# Autodesk Inventor assembly: Storage System Assembly
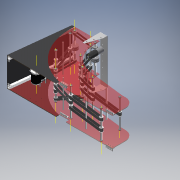
[picture p0: Inventor's stored thumbnail of the model, 180x180]
Saved by Autodesk Inventor 2019.4 (Build 234330000, 330)
## iProperties
Created: 2020-01-11
Part Number: Storage System Assembly
Document SubType Name: Assembly
Designer: admin
Mass: 8566.96 g
Surface Area: 28406.6 cm^2
Volume: 5013.1 cm^3
Density: 1.70891 g/cm^3
Author: admin
## Documents named in this file (37)
- C:\Users\admin\Desktop\FRC 2020 Engineering\GitHub\7738-2020\Storage system\Storage System Assembly.iam
- C:\Users\admin\Desktop\FRC 2020 Engineering\GitHub\7738-2020\Storage system\Turret Base Plate.ipt
- C:\Users\admin\Desktop\FRC 2020 Engineering\GitHub\7738-2020\Storage system\Storage Side Plate.ipt
- C:\Users\admin\Desktop\FRC 2020 Engineering\GitHub\7738-2020\CAD\Gearbox\F6800.ipt
- C:\Users\admin\Desktop\FRC 2020 Engineering\GitHub\7738-2020\Storage system\Storage System Assembly\Design Accelerator\Synchronous Belts Transmission1.iam
- C:\Users\admin\Desktop\FRC 2020 Engineering\GitHub\7738-2020\Storage system\Storage System Assembly\Design Accelerator\Synchronous Belts Transmission2.iam
- C:\Users\admin\Desktop\FRC 2020 Engineering\GitHub\7738-2020\Storage system\Storage System Assembly\Design Accelerator\Synchronous Belts Transmission3.iam
- C:\Users\admin\Desktop\FRC 2020 Engineering\GitHub\7738-2020\Storage system\Storage System Assembly\Design Accelerator\Synchronous Belts Transmission5.iam
- C:\Users\admin\Desktop\FRC 2020 Engineering\GitHub\7738-2020\Storage system\Storage System Assembly\Design Accelerator\Synchronous Belts Transmission6.iam
- C:\Users\admin\Desktop\FRC 2020 Engineering\GitHub\7738-2020\Storage system\Storage System Assembly\Design Accelerator\Synchronous Belts Transmission7.iam
- C:\Users\admin\Desktop\FRC 2020 Engineering\GitHub\7738-2020\Storage system\Storage System Assembly\Design Accelerator\Synchronous Belts Transmission8.iam
- C:\Users\admin\Desktop\FRC 2020 Engineering\GitHub\7738-2020\Storage system\Storage System Assembly\Design Accelerator\Synchronous Belts Transmission9.iam
- C:\Users\admin\Desktop\FRC 2020 Engineering\GitHub\7738-2020\Storage system\Complaint Wheel.ipt
- C:\Users\admin\Desktop\FRC 2020 Engineering\GitHub\7738-2020\Storage system\Belt Axle.ipt
- C:\Users\admin\Desktop\FRC 2020 Engineering\GitHub\7738-2020\Storage system\Storage System Assembly\Design Accelerator\Synchronous Belts Transmission4.iam
- C:\Users\admin\Desktop\FRC 2020 Engineering\GitHub\7738-2020\Storage system\Storage System Assembly\Design Accelerator\Synchronous Belts Transmission10.iam
- C:\Users\admin\Desktop\FRC 2020 Engineering\GitHub\7738-2020\Storage system\Storage System Assembly\Design Accelerator\Synchronous Belts Transmission11.iam
- C:\Users\admin\Desktop\FRC 2020 Engineering\GitHub\7738-2020\Storage system\Storage System Assembly\Design Accelerator\Synchronous Belts Transmission12.iam
- C:\Users\admin\Desktop\FRC 2020 Engineering\GitHub\7738-2020\Storage system\Storage Plate Spacer.ipt
- C:\Users\admin\Desktop\FRC 2020 Engineering\GitHub\7738-2020\Storage system\PC Plate Bracket.ipt
- C:\Users\admin\Desktop\FRC 2020 Engineering\GitHub\7738-2020\Storage system\Turret Support Extrusion.ipt
- C:\Users\admin\Desktop\FRC 2020 Engineering\GitHub\7738-2020\Storage system\Back PC Cover.ipt
- C:\Users\admin\Desktop\FRC 2020 Engineering\GitHub\7738-2020\Storage system\Side CFRP Cover.ipt
- C:\Users\admin\Desktop\FRC 2020 Engineering\GitHub\7738-2020\Storage system\Turret Drive Gear.ipt
- C:\Users\admin\Desktop\FRC 2020 Engineering\GitHub\7738-2020\Storage system\Sport Gearbox\775pro_217-4347.ipt
- C:\Users\admin\Desktop\FRC 2020 Engineering\GitHub\7738-2020\Storage system\775 16 reduction Gearbox.ipt
- C:\Users\admin\Desktop\FRC 2020 Engineering\GitHub\7738-2020\Turret\Turret Support Brace.ipt
- C:\Users\admin\Desktop\FRC 2020 Engineering\GitHub\7738-2020\Storage system\Brace.ipt
- C:\Users\admin\Desktop\FRC 2020 Engineering\GitHub\7738-2020\Storage system\Intake Motor Mount.ipt
- C:\Users\admin\Desktop\FRC 2020 Engineering\GitHub\7738-2020\Turret\Mini CIM\Mini_CIM_Motor_217-3371.ipt
- C:\Users\admin\Desktop\FRC 2020 Engineering\GitHub\7738-2020\Storage system\Storage System Assembly\Design Accelerator\Synchronous Belts Transmission13.iam
- C:\Users\admin\Desktop\FRC 2020 Engineering\GitHub\7738-2020\Storage system\Spacer.ipt
- C:\Users\admin\Desktop\FRC 2020 Engineering\GitHub\7738-2020\Storage system\Storage System Assembly\Design Accelerator\Synchronous Belts Transmission14.iam
- C:\Users\admin\Desktop\FRC 2020 Engineering\GitHub\7738-2020\Storage system\Storage System Assembly\Design Accelerator\Synchronous Belts Transmission15.iam
- C:\Users\admin\Desktop\FRC 2020 Engineering\GitHub\7738-2020\Storage system\Storage Shooter Axle.ipt
- C:\Users\admin\Desktop\FRC 2020 Engineering\GitHub\7738-2020\Storage system\Storage System Assembly\Design Accelerator\Spur Gears1.iam
- C:\Users\admin\Desktop\FRC 2020 Engineering\GitHub\7738-2020\Storage system\Storage System Assembly\Design Accelerator\Synchronous Belts Transmission16.iam
## Components (98 placed, 21 different names)
1. Turret Base Plate:1 — Mate:1, Mate:3, Mate:4, Flush:1, Mate:5, Mate:8, Mate:9, Angle:1, Mate:107, Mate:108, Mate:110, Mate:119, Mate:120, Mate:121, Mate:122, Mate:125, Mate:126, Flush:16, Mate:132, Mate:135
2. Storage Side Plate:1 — Mate:1, Mate:7, Mate:8, Mate:10, Mate:11, Mate:12, Mate:13, Mate:14, Mate:15, Mate:16, Mate:17, Mate:18, Mate:19, Mate:20, Mate:21, Mate:22, Mate:23, Mate:24, Mate:25, Mate:26, Mate:27, Mate:28, Mate:29, Mate:30, Mate:31, Mate:32, Mate:33, Symmetry:1, Mate:75, Mate:93, Mate:94, Mate:95, Mate:96, Mate:97, Mate:98, Mate:99, Mate:100, Mate:101, Flush:4, Mate:102, Mate:105, Flush:6, Flush:7, Mate:107, Mate:111, Flush:11, Mate:114, Mate:115, Flush:12, Flush:13, Mate:137, Mate:138, Mate:139, Mate:147, Mate:148, Mate:149, Mate:150, Mate:169, Mate:170, Mate:171
3. Storage Side Plate:2 — Mate:5, Mate:7, Mate:9, Symmetry:1, Mate:41, Mate:42, Mate:43, Mate:44, Mate:45, Mate:46, Mate:47, Mate:48, Mate:49, Mate:50, Mate:51, Mate:52, Mate:53, Mate:54, Mate:55, Mate:56, Mate:57, Mate:58, Mate:59, Mate:60, Mate:61, Mate:62, Mate:63, Mate:64, Mate:85, Mate:86, Mate:87, Mate:88, Mate:89, Mate:90, Mate:91, Mate:92, Mate:103, Mate:104, Flush:5, Mate:106, Flush:8, Flush:9, Mate:109, Flush:10, Mate:113, Mate:116, Flush:14, Flush:15, Mate:157, Mate:162, Mate:163
4. Synchronous Belts Transmission:1 [sub-assembly] — Mate:66
5. Synchronous Belts Transmission:2 [sub-assembly]
6. Synchronous Belts Transmission:3 [sub-assembly]
7. Synchronous Belts Transmission:4 [sub-assembly]
8. Synchronous Belts Transmission:5 [sub-assembly]
9. Synchronous Belts Transmission:6 [sub-assembly]
10. Synchronous Belts Transmission:7 [sub-assembly]
11. Synchronous Belts Transmission:8 [sub-assembly]
12. F6800:11 — Mate:30, Mate:32, Mate:34
13. F6800:12 — Mate:31, Mate:33, Mate:39
14. Complaint Wheel:1 — Mate:34, Mate:35, Mate:36, Flush:3
15. Complaint Wheel:2 — Mate:35, Mate:36, Mate:40
16. Complaint Wheel:3 — Flush:3
17. Complaint Wheel:4 — Mate:39
18. Synchronous Belts Transmission:9 [sub-assembly]
19. Synchronous Belts Transmission:10 [sub-assembly]
20. Synchronous Belts Transmission:11 [sub-assembly]
21. Synchronous Belts Transmission:12 [sub-assembly]
22. Storage Plate Spacer:1 — Mate:85, Mate:93
23. Storage Plate Spacer:2 — Mate:89, Mate:100
24. Storage Plate Spacer:3 — Mate:90, Mate:99
25. Storage Plate Spacer:4 — Mate:91, Mate:98
26. Storage Plate Spacer:5 — Mate:92, Mate:97
27. Storage Plate Spacer:6 — Mate:88, Mate:96
28. Storage Plate Spacer:7 — Mate:87, Mate:95
29. Storage Plate Spacer:8 — Mate:86, Mate:94
30. PC Plate Bracket:1 — Mate:101, Flush:4, Mate:102
31. PC Plate Bracket:2 — Mate:103, Mate:104, Flush:5
32. PC Plate Bracket:3 — Mate:105, Flush:6, Flush:7
33. PC Plate Bracket:4 — Mate:106, Flush:8, Flush:9
34. Turret Support Extrusion:1 — Mate:108, Mate:109, Flush:10, Mate:112, Mate:127, Flush:17, Mate:128, Mate:131, Mate:133
35. Turret Support Extrusion:2 — Mate:110, Mate:111, Flush:11, Mate:129, Flush:18, Mate:130, Mate:134, Mate:136
36. Back PC Cover:1 — Mate:112, Mate:113, Mate:114
37. Side CFRP Cover:1 — Mate:115, Flush:12, Flush:13
38. Side CFRP Cover:2 — Mate:116, Flush:14, Flush:15
39. Turret Drive Gear:1 — Mate:119, Mate:120
40. 775pro_217-4347:1 — Mate:123, Mate:124
41. 775 16 reduction Gearbox:1 — Mate:121, Mate:122, Mate:123, Mate:124
42. Turret Support Brace:1 — Mate:125, Mate:126, Flush:16
43. Brace:1 — Mate:127, Flush:17, Mate:128
44. Brace:2 — Mate:129, Flush:18, Mate:130
45. Brace:3 — Mate:131, Mate:132, Mate:133
46. Brace:4 — Mate:134, Mate:135, Mate:136
47. Intake Motor Mount:1 — Mate:137, Mate:138, Mate:139, Mate:140, Mate:142, Mate:143, Mate:144, Mate:145, Mate:146
48. Mini_CIM_Motor_217-3371:1 — Mate:140, Mate:142
49. Synchronous Belts Transmission:13 [sub-assembly]
50. Spacer:1 — Mate:143, Mate:150
51. Spacer:2 — Mate:146, Mate:149
52. Spacer:3 — Mate:144, Mate:147
53. Spacer:4 — Mate:145, Mate:148
54. Synchronous Belts Transmission:14 [sub-assembly]
55. Intake Motor Mount:2 — Mate:157, Mate:158, Mate:159, Mate:160, Mate:161
56. Mini_CIM_Motor_217-3371:2
57. Spacer:5 — Mate:160
58. Spacer:6 — Mate:161
59. Spacer:7 — Mate:158, Mate:163
60. Spacer:8 — Mate:159, Mate:162
61. Synchronous Belts Transmission:15 [sub-assembly]
62. Storage Shooter Axle:1 — Mate:166, Mate:167, Mate:168
63. Storage Shooter Axle:2 — Mate:164, Mate:165
64. Spur Gears:1 [sub-assembly] — Mate:168, Mate:169
65. Synchronous Belts Transmission:16 [sub-assembly]
66. F6800:25 — Mate:170, Mate:171
67. Belt Axle:10 — Mate:74, Mate:84
68. Belt Axle:9 — Mate:73, Mate:83
69. Belt Axle:8 — Mate:72, Mate:82
70. Belt Axle:7 — Mate:71, Mate:81
71. Belt Axle:6 — Mate:70, Mate:80
72. Belt Axle:5 — Mate:69, Mate:75
73. Belt Axle:4 — Mate:68, Mate:76
74. Belt Axle:3 — Mate:67, Mate:77
75. Belt Axle:2 — Mate:66, Mate:78
76. Belt Axle:1 — Mate:65, Mate:79
77. F6800:10 — Mate:19, Mate:25, Mate:70, Mate:80
78. F6800:9 — Mate:18, Mate:26, Mate:71, Mate:81
79. F6800:7 — Mate:16, Mate:28, Mate:73, Mate:83
80. F6800:8 — Mate:17, Mate:27, Mate:72, Mate:82
81. F6800:6 — Mate:15, Mate:29, Mate:74, Mate:84
82. F6800:5 — Mate:14, Mate:24, Mate:69
83. F6800:4 — Mate:13, Mate:23, Mate:68, Mate:76
84. F6800:3 — Mate:12, Mate:22, Mate:67, Mate:77
85. F6800:2 — Mate:11, Mate:21, Mate:78
86. F6800:1 — Mate:10, Mate:20, Mate:65, Mate:79
87. F6800:24 — Mate:52, Mate:64
88. F6800:23 — Mate:51, Mate:63
89. F6800:22 — Mate:49, Mate:61
90. F6800:21 — Mate:50, Mate:62
91. F6800:20 — Mate:48, Mate:60
92. F6800:19 — Mate:47, Mate:59
93. F6800:18 — Mate:46, Mate:57
94. F6800:17 — Mate:45, Mate:58
95. F6800:16 — Mate:44, Mate:55
96. F6800:15 — Mate:42, Mate:53, Mate:166, Mate:167
97. F6800:13 — Mate:41, Mate:54, Mate:164, Mate:165
98. F6800:14 — Mate:43, Mate:56
## Relationships (185: Mate 166, Flush 17, Angle 1, Symmetry 1)
- Mate:1: Turret Base Plate:1 ↔ Storage Side Plate:1
- Mate:3: Turret Base Plate:1
- Mate:4: Turret Base Plate:1
- Flush:1: Turret Base Plate:1
- Mate:5: Turret Base Plate:1 ↔ Storage Side Plate:2
- Mate:7: Storage Side Plate:1 ↔ Storage Side Plate:2
- Mate:8 (3 mm): Turret Base Plate:1 ↔ Storage Side Plate:1
- Mate:9 (3 mm): Turret Base Plate:1 ↔ Storage Side Plate:2
- Mate:10: Storage Side Plate:1 ↔ F6800:1
- Mate:11: Storage Side Plate:1 ↔ F6800:2
- Mate:12: Storage Side Plate:1 ↔ F6800:3
- Mate:13: Storage Side Plate:1 ↔ F6800:4
- Mate:14: Storage Side Plate:1 ↔ F6800:5
- Mate:15: Storage Side Plate:1 ↔ F6800:6
- Mate:16: Storage Side Plate:1 ↔ F6800:7
- Mate:17: Storage Side Plate:1 ↔ F6800:8
- Mate:18: Storage Side Plate:1 ↔ F6800:9
- Mate:19: Storage Side Plate:1 ↔ F6800:10
- Mate:20 (0.2 mm): Storage Side Plate:1 ↔ F6800:1
- Mate:21 (0.2 mm): Storage Side Plate:1 ↔ F6800:2
- Mate:22 (0.2 mm): Storage Side Plate:1 ↔ F6800:3
- Mate:23 (0.2 mm): Storage Side Plate:1 ↔ F6800:4
- Mate:24 (0.2 mm): Storage Side Plate:1 ↔ F6800:5
- Mate:25 (0.2 mm): Storage Side Plate:1 ↔ F6800:10
- Mate:26 (0.2 mm): Storage Side Plate:1 ↔ F6800:9
- Mate:27 (0.2 mm): Storage Side Plate:1 ↔ F6800:8
- Mate:28 (0.2 mm): Storage Side Plate:1 ↔ F6800:7
- Mate:29 (0.2 mm): Storage Side Plate:1 ↔ F6800:6
- Angle:1 (180 deg): Turret Base Plate:1
- Mate:30: Storage Side Plate:1 ↔ F6800:11
- Mate:31: Storage Side Plate:1 ↔ F6800:12
- Mate:32 (0.2 mm): Storage Side Plate:1 ↔ F6800:11
- Mate:33 (0.2 mm): Storage Side Plate:1 ↔ F6800:12
- Mate:34: F6800:11 ↔ Complaint Wheel:1
- Mate:35: Complaint Wheel:1 ↔ Complaint Wheel:2
- Mate:36 (1 mm): Complaint Wheel:1 ↔ Complaint Wheel:2
- [Mate]: Complaint Wheel:3 ↔ Complaint Wheel:4
- [Mate] (1 mm): Complaint Wheel:3 ↔ Complaint Wheel:4
- Mate:39: F6800:12 ↔ Complaint Wheel:4
- Flush:3: Complaint Wheel:1 ↔ Complaint Wheel:3
- Symmetry:1: Storage Side Plate:1 ↔ Storage Side Plate:2
- Mate:40 (0.5 mm): Complaint Wheel:2
- Mate:41: Storage Side Plate:2 ↔ F6800:13
- Mate:42: Storage Side Plate:2 ↔ F6800:15
- Mate:43: Storage Side Plate:2 ↔ F6800:14
- Mate:44: Storage Side Plate:2 ↔ F6800:16
- Mate:45: Storage Side Plate:2 ↔ F6800:17
- Mate:46: Storage Side Plate:2 ↔ F6800:18
- Mate:47: Storage Side Plate:2 ↔ F6800:19
- Mate:48: Storage Side Plate:2 ↔ F6800:20
- Mate:49: Storage Side Plate:2 ↔ F6800:22
- Mate:50: Storage Side Plate:2 ↔ F6800:21
- Mate:51: Storage Side Plate:2 ↔ F6800:23
- Mate:52: Storage Side Plate:2 ↔ F6800:24
- Mate:53 (0.2 mm): Storage Side Plate:2 ↔ F6800:15
- Mate:54 (0.2 mm): Storage Side Plate:2 ↔ F6800:13
- Mate:55 (0.2 mm): Storage Side Plate:2 ↔ F6800:16
- Mate:56 (0.2 mm): Storage Side Plate:2 ↔ F6800:14
- Mate:57 (0.2 mm): Storage Side Plate:2 ↔ F6800:18
- Mate:58 (0.2 mm): Storage Side Plate:2 ↔ F6800:17
- Mate:59 (0.2 mm): Storage Side Plate:2 ↔ F6800:19
- Mate:60 (0.2 mm): Storage Side Plate:2 ↔ F6800:20
- Mate:61 (0.2 mm): Storage Side Plate:2 ↔ F6800:22
- Mate:62 (0.2 mm): Storage Side Plate:2 ↔ F6800:21
- Mate:63 (0.2 mm): Storage Side Plate:2 ↔ F6800:23
- Mate:64 (0.2 mm): Storage Side Plate:2 ↔ F6800:24
- Mate:65: Belt Axle:1 ↔ F6800:1
- Mate:66: Synchronous Belts Transmission:1 ↔ Belt Axle:2
- Mate:67: Belt Axle:3 ↔ F6800:3
- Mate:68: Belt Axle:4 ↔ F6800:4
- Mate:69: Belt Axle:5 ↔ F6800:5
- Mate:70: Belt Axle:6 ↔ F6800:10
- Mate:71: Belt Axle:7 ↔ F6800:9
- Mate:72: Belt Axle:8 ↔ F6800:8
- Mate:73: Belt Axle:9 ↔ F6800:7
- Mate:74: Belt Axle:10 ↔ F6800:6
- Mate:75 (0.2 mm): Storage Side Plate:1 ↔ Belt Axle:5
- Mate:76 (0.2 mm): Belt Axle:4 ↔ F6800:4
- Mate:77 (0.2 mm): Belt Axle:3 ↔ F6800:3
- Mate:78 (0.2 mm): Belt Axle:2 ↔ F6800:2
- Mate:79 (0.2 mm): Belt Axle:1 ↔ F6800:1
- Mate:80 (0.2 mm): Belt Axle:6 ↔ F6800:10
- Mate:81 (0.2 mm): Belt Axle:7 ↔ F6800:9
- Mate:82 (0.2 mm): Belt Axle:8 ↔ F6800:8
- Mate:83 (0.2 mm): Belt Axle:9 ↔ F6800:7
- Mate:84 (0.2 mm): Belt Axle:10 ↔ F6800:6
- Mate:85: Storage Side Plate:2 ↔ Storage Plate Spacer:1
- Mate:86: Storage Side Plate:2 ↔ Storage Plate Spacer:8
- Mate:87: Storage Side Plate:2 ↔ Storage Plate Spacer:7
- Mate:88: Storage Side Plate:2 ↔ Storage Plate Spacer:6
- Mate:89: Storage Side Plate:2 ↔ Storage Plate Spacer:2
- Mate:90: Storage Side Plate:2 ↔ Storage Plate Spacer:3
- Mate:91: Storage Side Plate:2 ↔ Storage Plate Spacer:4
- Mate:92: Storage Side Plate:2 ↔ Storage Plate Spacer:5
- Mate:93 (0.2 mm): Storage Side Plate:1 ↔ Storage Plate Spacer:1
- Mate:94 (0.2 mm): Storage Side Plate:1 ↔ Storage Plate Spacer:8
- Mate:95 (0.2 mm): Storage Side Plate:1 ↔ Storage Plate Spacer:7
- Mate:96 (0.2 mm): Storage Side Plate:1 ↔ Storage Plate Spacer:6
- Mate:97 (0.2 mm): Storage Side Plate:1 ↔ Storage Plate Spacer:5
- Mate:98 (0.2 mm): Storage Side Plate:1 ↔ Storage Plate Spacer:4
- Mate:99 (0.2 mm): Storage Side Plate:1 ↔ Storage Plate Spacer:3
- Mate:100 (0.2 mm): Storage Side Plate:1 ↔ Storage Plate Spacer:2
- Mate:101: Storage Side Plate:1 ↔ PC Plate Bracket:1
- Flush:4: Storage Side Plate:1 ↔ PC Plate Bracket:1
- Mate:102 (3 mm): Storage Side Plate:1 ↔ PC Plate Bracket:1
- Mate:103: Storage Side Plate:2 ↔ PC Plate Bracket:2
- Mate:104 (3 mm): Storage Side Plate:2 ↔ PC Plate Bracket:2
- Flush:5: Storage Side Plate:2 ↔ PC Plate Bracket:2
- Mate:105: Storage Side Plate:1 ↔ PC Plate Bracket:3
- Flush:6: Storage Side Plate:1 ↔ PC Plate Bracket:3
- Flush:7: Storage Side Plate:1 ↔ PC Plate Bracket:3
- Mate:106: Storage Side Plate:2 ↔ PC Plate Bracket:4
- Flush:8: Storage Side Plate:2 ↔ PC Plate Bracket:4
- Flush:9: Storage Side Plate:2 ↔ PC Plate Bracket:4
- Mate:107: Turret Base Plate:1 ↔ Storage Side Plate:1
- Mate:108: Turret Base Plate:1 ↔ Turret Support Extrusion:1
- Mate:109: Storage Side Plate:2 ↔ Turret Support Extrusion:1
- Flush:10 (3 mm): Storage Side Plate:2 ↔ Turret Support Extrusion:1
- Mate:110: Turret Base Plate:1 ↔ Turret Support Extrusion:2
- Mate:111: Storage Side Plate:1 ↔ Turret Support Extrusion:2
- Flush:11 (5 mm): Storage Side Plate:1 ↔ Turret Support Extrusion:2
- Mate:112: Turret Support Extrusion:1 ↔ Back PC Cover:1
- Mate:113 (1 mm): Storage Side Plate:2 ↔ Back PC Cover:1
- Mate:114: Storage Side Plate:1 ↔ Back PC Cover:1
- Mate:115: Storage Side Plate:1 ↔ Side CFRP Cover:1
- Flush:12: Storage Side Plate:1 ↔ Side CFRP Cover:1
- Flush:13: Storage Side Plate:1 ↔ Side CFRP Cover:1
- Mate:116: Storage Side Plate:2 ↔ Side CFRP Cover:2
- Flush:14: Storage Side Plate:2 ↔ Side CFRP Cover:2
- Flush:15: Storage Side Plate:2 ↔ Side CFRP Cover:2
- Mate:119: Turret Base Plate:1 ↔ Turret Drive Gear:1
- Mate:120 (10 mm): Turret Base Plate:1 ↔ Turret Drive Gear:1
- Mate:121: Turret Base Plate:1 ↔ 775 16 reduction Gearbox:1
- Mate:122 (5 mm): Turret Base Plate:1 ↔ 775 16 reduction Gearbox:1
- Mate:123: 775pro_217-4347:1 ↔ 775 16 reduction Gearbox:1
- Mate:124: 775pro_217-4347:1 ↔ 775 16 reduction Gearbox:1
- Mate:125: Turret Base Plate:1 ↔ Turret Support Brace:1
- Mate:126 (0.5 mm): Turret Base Plate:1 ↔ Turret Support Brace:1
- Flush:16 (-70 mm): Turret Base Plate:1 ↔ Turret Support Brace:1
- Mate:127: Turret Support Extrusion:1 ↔ Brace:1
- Flush:17: Turret Support Extrusion:1 ↔ Brace:1
- Mate:128 (-0.5 mm): Turret Support Extrusion:1 ↔ Brace:1
- Mate:129: Turret Support Extrusion:2 ↔ Brace:2
- Flush:18: Turret Support Extrusion:2 ↔ Brace:2
- Mate:130 (-0.5 mm): Turret Support Extrusion:2 ↔ Brace:2
- Mate:131: Turret Support Extrusion:1 ↔ Brace:3
- Mate:132: Turret Base Plate:1 ↔ Brace:3
- Mate:133 (-0.5 mm): Turret Support Extrusion:1 ↔ Brace:3
- Mate:134: Turret Support Extrusion:2 ↔ Brace:4
- Mate:135: Turret Base Plate:1 ↔ Brace:4
- Mate:136 (-0.5 mm): Turret Support Extrusion:2 ↔ Brace:4
- Mate:137: Storage Side Plate:1 ↔ Intake Motor Mount:1
- Mate:138: Storage Side Plate:1 ↔ Intake Motor Mount:1
- Mate:139 (35 mm): Storage Side Plate:1 ↔ Intake Motor Mount:1
- Mate:140: Intake Motor Mount:1 ↔ Mini_CIM_Motor_217-3371:1
- Mate:142: Intake Motor Mount:1 ↔ Mini_CIM_Motor_217-3371:1
- Mate:143: Intake Motor Mount:1 ↔ Spacer:1
- Mate:144: Intake Motor Mount:1 ↔ Spacer:3
- Mate:145: Intake Motor Mount:1 ↔ Spacer:4
- Mate:146: Intake Motor Mount:1 ↔ Spacer:2
- Mate:147: Storage Side Plate:1 ↔ Spacer:3
- Mate:148: Storage Side Plate:1 ↔ Spacer:4
- Mate:149: Storage Side Plate:1 ↔ Spacer:2
- Mate:150: Storage Side Plate:1 ↔ Spacer:1
- [Mate]: Intake Motor Mount:2 ↔ Mini_CIM_Motor_217-3371:2
- [Mate]: Intake Motor Mount:2 ↔ Mini_CIM_Motor_217-3371:2
- [Mate]: Intake Motor Mount:2 ↔ Spacer:5
- [Mate]: Intake Motor Mount:2 ↔ Spacer:7
- [Mate]: Intake Motor Mount:2 ↔ Spacer:8
- [Mate]: Intake Motor Mount:2 ↔ Spacer:6
- Mate:157 (35 mm): Storage Side Plate:2 ↔ Intake Motor Mount:2
- Mate:158: Intake Motor Mount:2 ↔ Spacer:7
- Mate:159: Intake Motor Mount:2 ↔ Spacer:8
- Mate:160: Intake Motor Mount:2 ↔ Spacer:5
- Mate:161: Intake Motor Mount:2 ↔ Spacer:6
- Mate:162: Storage Side Plate:2 ↔ Spacer:8
- Mate:163: Storage Side Plate:2 ↔ Spacer:7
- Mate:164: Storage Shooter Axle:2 ↔ F6800:13
- Mate:165 (0.2 mm): Storage Shooter Axle:2 ↔ F6800:13
- Mate:166: Storage Shooter Axle:1 ↔ F6800:15
- Mate:167 (0.2 mm): Storage Shooter Axle:1 ↔ F6800:15
- Mate:168: Storage Shooter Axle:1 ↔ Spur Gears:1
- Mate:169 (30 mm): Storage Side Plate:1 ↔ Spur Gears:1
- Mate:170: Storage Side Plate:1 ↔ F6800:25
- Mate:171 (0.2 mm): Storage Side Plate:1 ↔ F6800:25
## Named parameters: d40_d38 = 0 mm, d41_d39 = 1 mm, d180_d174 = 0 mm, d181_d172 = 0 mm, d182_d173 = 0 mm, d183_d175 = 0 mm, d184_d169 = 0 mm, d185_d171 = 0 mm
